# Autodesk Inventor assembly: MS-1
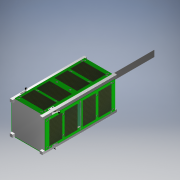
[picture p0: Inventor's stored thumbnail of the model, 180x180]
Saved by Autodesk Inventor 2022.3 (Build 263350000, 350)
## iProperties
Created: 2021-04-30
Part Number: MS-1
Document SubType Name: Assembly
Designer: Bowen O'Steen
Mass: 1447.72 g
Surface Area: 6988.67 cm^2
Volume: 630.884 cm^3
Density: 2.29475 g/cm^3
Author: Bowen O'Steen
## Documents named in this file (13)
- C:\Users\gwhen\OneDrive\Documents\Vault\Engineering Data\MemeSat\Assembly\MS-1.iam
- C:\Users\gwhen\OneDrive\Documents\Vault\Engineering Data\MemeSat\Assembly\boardstack.iam
- C:\Users\gwhen\OneDrive\Documents\Vault\Engineering Data\MemeSat\Assembly\FR-01assembled.iam
- C:\Users\gwhen\OneDrive\Documents\Vault\Engineering Data\MemeSat\Assembly\FR-04assembled.iam
- C:\Users\gwhen\OneDrive\Documents\Vault\Engineering Data\MemeSat\Assembly\FR-02assembled.iam
- C:\Users\gwhen\OneDrive\Documents\Vault\Engineering Data\MemeSat\Assembly\FR-03assembled.iam
- C:\Users\gwhen\OneDrive\Documents\Vault\Engineering Data\MemeSat\Assembly\FR-05assembled.iam
- C:\Users\gwhen\OneDrive\Documents\Vault\Engineering Data\MemeSat\Assembly\FR-06assembled.iam
- C:\Users\gwhen\OneDrive\Desktop\Vault\Designs\MEMESat\MemeSat\Engineering Data\MemeSat\Fasteners\92949A106_18-8 Stainless Steel Button Head Hex Drive Screw.ipt
- C:\Users\gwhen\OneDrive\Desktop\Vault\Designs\MEMESat\MemeSat\Engineering Data\MemeSat\Switches\ss-01gl2.ipt
- C:\Users\gwhen\OneDrive\Desktop\Vault\Designs\MEMESat\MemeSat\Engineering Data\MemeSat\Fasteners\92095A455_Button Head Hex Drive Screw.ipt
- C:\Users\gwhen\OneDrive\Desktop\Vault\Designs\MEMESat\MemeSat\Engineering Data\MemeSat\Fasteners\91828A111_18-8 Stainless Steel Hex Nut.ipt
- C:\Users\gwhen\OneDrive\Desktop\Vault\Designs\MEMESat\MemeSat\Engineering Data\MemeSat\Fasteners\90730A005.ipt
## Components (135 placed, 12 different names)
1. FR-01assembled:1 [sub-assembly] — Mate:1, Mate:2, Flush:1, Mate:3, Mate:4, Mate:5, Mate:6, Mate:7, Mate:8, Mate:13, Mate:14, Mate:15, Mate:16, Mate:47, Mate:49
2. FR-02assembled:1 [sub-assembly] — Mate:9, Mate:10, Mate:11, Mate:12, Mate:17, Mate:25, Mate:35, Mate:37, Mate:43, Mate:64, Mate:65, Mate:66, Mate:67, Mate:68, Mate:69, Mate:70, Mate:71, Mate:72, Mate:73, Mate:74, Mate:75, Mate:76, Mate:77, Mate:78, Mate:79, Mate:362, Mate:363, Mate:364, Mate:365, Mate:370, Mate:371, Mate:372, Mate:373, Mate:374, Mate:377, Mate:378, Mate:379, Mate:380, Mate:381, Mate:382, Mate:383
3. FR-03assembled:1 [sub-assembly] — Mate:6, Mate:7, Mate:8, Mate:19, Mate:20, Mate:21, Mate:22, Mate:23, Mate:24, Mate:26, Mate:59, Mate:60, Mate:61, Mate:160, Mate:161, Mate:162, Mate:163, Mate:164, Mate:165, Mate:166, Mate:167, Mate:229, Mate:230, Mate:231, Mate:244, Mate:245, Mate:270, Mate:271, Mate:302, Mate:303, Mate:308, Mate:309, Mate:320, Mate:322, Mate:334, Mate:335, Mate:358, Mate:359
4. FR-04assembled:1 [sub-assembly] — Mate:3, Mate:4, Mate:5, Mate:9, Mate:10, Mate:11, Mate:27, Mate:28, Mate:29, Mate:30, Mate:31, Mate:32, Mate:33, Mate:34, Mate:152, Mate:153, Mate:154, Mate:155, Mate:156, Mate:157, Mate:158, Mate:159, Mate:209, Mate:211, Mate:232, Mate:233, Mate:234, Mate:261, Mate:262, Mate:276, Mate:277, Mate:304, Mate:305, Mate:306, Mate:307, Mate:318, Mate:319, Mate:343, Mate:345, Mate:354, Mate:355
5. FR-05assembled:1 [sub-assembly] — Mate:15, Mate:16, Mate:17, Mate:36, Mate:38, Mate:39, Mate:40, Mate:41, Mate:42, Mate:51, Mate:52, Mate:53, Mate:54, Mate:57, Mate:144, Mate:145, Mate:146, Mate:147, Mate:148, Mate:149, Mate:150, Mate:151, Mate:225, Mate:235, Mate:236, Mate:237, Mate:241, Mate:274, Mate:275, Mate:298, Mate:299, Mate:300, Mate:301, Mate:314, Mate:315, Mate:330, Mate:331, Mate:346, Mate:347
6. FR-06assembled:1 [sub-assembly] — Mate:12, Mate:13, Mate:14, Mate:44, Mate:45, Mate:46, Mate:48, Mate:50, Mate:168, Mate:169, Mate:170, Mate:171, Mate:172, Mate:173, Mate:174, Mate:175, Mate:213, Mate:215, Mate:226, Mate:227, Mate:228, Mate:242, Mate:243, Mate:272, Mate:273, Mate:310, Mate:311, Mate:312, Mate:313, Mate:316, Mate:317, Mate:332, Mate:333, Mate:348, Mate:349
7. boardstack:1 [sub-assembly] — Mate:55, Mate:56, Mate:57, Mate:58, Mate:62, Mate:63, Mate:96, Mate:97, Mate:98, Mate:99, Mate:100, Mate:101, Mate:102, Mate:103, Mate:104, Mate:105, Mate:106, Mate:107, Mate:108, Mate:109, Mate:110, Mate:111, Mate:208, Mate:210, Mate:212, Mate:214, Mate:278, Mate:279, Mate:280, Mate:281, Mate:282, Mate:283, Mate:284, Mate:285
8. 92949A106_18-8 Stainless Steel Button Head Hex Drive Screw:2 — Mate:21, Mate:22
9. 92949A106_18-8 Stainless Steel Button Head Hex Drive Screw:3 — Mate:19, Mate:20
10. 92949A106_18-8 Stainless Steel Button Head Hex Drive Screw:4 — Mate:23, Mate:24
11. 92949A106_18-8 Stainless Steel Button Head Hex Drive Screw:5 — Mate:47, Mate:48
12. 92949A106_18-8 Stainless Steel Button Head Hex Drive Screw:6 — Mate:25, Mate:26
13. 92949A106_18-8 Stainless Steel Button Head Hex Drive Screw:7 — Mate:27, Mate:28
14. 92949A106_18-8 Stainless Steel Button Head Hex Drive Screw:8 — Mate:31, Mate:32
15. 92949A106_18-8 Stainless Steel Button Head Hex Drive Screw:9 — Mate:33, Mate:34
16. 92949A106_18-8 Stainless Steel Button Head Hex Drive Screw:10 — Mate:29, Mate:30
17. 92949A106_18-8 Stainless Steel Button Head Hex Drive Screw:11 — Mate:35, Mate:36
18. 92949A106_18-8 Stainless Steel Button Head Hex Drive Screw:12 — Mate:39, Mate:40
19. 92949A106_18-8 Stainless Steel Button Head Hex Drive Screw:13 — Mate:37, Mate:38
20. 92949A106_18-8 Stainless Steel Button Head Hex Drive Screw:14 — Mate:41, Mate:42
21. 92949A106_18-8 Stainless Steel Button Head Hex Drive Screw:15 — Mate:43, Mate:44
22. 92949A106_18-8 Stainless Steel Button Head Hex Drive Screw:16 — Mate:45, Mate:46
23. 92949A106_18-8 Stainless Steel Button Head Hex Drive Screw:17 — Mate:49, Mate:50
24. 92949A106_18-8 Stainless Steel Button Head Hex Drive Screw:18 — Mate:58, Mate:61, Mate:62
25. 92949A106_18-8 Stainless Steel Button Head Hex Drive Screw:19 — Mate:59, Mate:60, Mate:63
26. 92949A106_18-8 Stainless Steel Button Head Hex Drive Screw:20 — Mate:51, Mate:52, Mate:55
27. 92949A106_18-8 Stainless Steel Button Head Hex Drive Screw:21 — Mate:53, Mate:54, Mate:56
28. 92949A106_18-8 Stainless Steel Button Head Hex Drive Screw:22 — Mate:67, Mate:71
29. 92949A106_18-8 Stainless Steel Button Head Hex Drive Screw:23 — Mate:64, Mate:68
30. 92949A106_18-8 Stainless Steel Button Head Hex Drive Screw:24 — Mate:65, Mate:69, Mate:375
31. 92949A106_18-8 Stainless Steel Button Head Hex Drive Screw:25 — Mate:66, Mate:70, Mate:376
32. 92949A106_18-8 Stainless Steel Button Head Hex Drive Screw:26 — Mate:75, Mate:76, Mate:368
33. 92949A106_18-8 Stainless Steel Button Head Hex Drive Screw:27 — Mate:74, Mate:79, Mate:367
34. 92949A106_18-8 Stainless Steel Button Head Hex Drive Screw:28 — Mate:72, Mate:78, Mate:366
35. 92949A106_18-8 Stainless Steel Button Head Hex Drive Screw:29 — Mate:73, Mate:77, Mate:369
36. 92949A106_18-8 Stainless Steel Button Head Hex Drive Screw:30 — Mate:96, Mate:97
37. 92949A106_18-8 Stainless Steel Button Head Hex Drive Screw:31 — Mate:98, Mate:99
38. 92949A106_18-8 Stainless Steel Button Head Hex Drive Screw:32 — Mate:100, Mate:101
39. 92949A106_18-8 Stainless Steel Button Head Hex Drive Screw:33 — Mate:102, Mate:103
40. 92949A106_18-8 Stainless Steel Button Head Hex Drive Screw:34 — Mate:108, Mate:109
41. 92949A106_18-8 Stainless Steel Button Head Hex Drive Screw:35 — Mate:110, Mate:111
42. 92949A106_18-8 Stainless Steel Button Head Hex Drive Screw:36 — Mate:104, Mate:105
43. 92949A106_18-8 Stainless Steel Button Head Hex Drive Screw:37 — Mate:106, Mate:107
44. 92949A106_18-8 Stainless Steel Button Head Hex Drive Screw:38 — Mate:147, Mate:150, Mate:353
45. 92949A106_18-8 Stainless Steel Button Head Hex Drive Screw:39 — Mate:146, Mate:151, Mate:352
46. 92949A106_18-8 Stainless Steel Button Head Hex Drive Screw:40 — Mate:145, Mate:149, Mate:337
47. 92949A106_18-8 Stainless Steel Button Head Hex Drive Screw:41 — Mate:144, Mate:148, Mate:339
48. 92949A106_18-8 Stainless Steel Button Head Hex Drive Screw:42 — Mate:155, Mate:156, Mate:357
49. 92949A106_18-8 Stainless Steel Button Head Hex Drive Screw:43 — Mate:154, Mate:157, Mate:356
50. 92949A106_18-8 Stainless Steel Button Head Hex Drive Screw:44 — Mate:153, Mate:158, Mate:344
51. 92949A106_18-8 Stainless Steel Button Head Hex Drive Screw:45 — Mate:152, Mate:159, Mate:338
52. 92949A106_18-8 Stainless Steel Button Head Hex Drive Screw:46 — Mate:160, Mate:165, Mate:342
53. 92949A106_18-8 Stainless Steel Button Head Hex Drive Screw:47 — Mate:161, Mate:166, Mate:341
54. 92949A106_18-8 Stainless Steel Button Head Hex Drive Screw:48 — Mate:162, Mate:167, Mate:361
55. 92949A106_18-8 Stainless Steel Button Head Hex Drive Screw:49 — Mate:163, Mate:164, Mate:360
56. 92949A106_18-8 Stainless Steel Button Head Hex Drive Screw:50 — Mate:170, Mate:173, Mate:350
57. 92949A106_18-8 Stainless Steel Button Head Hex Drive Screw:51 — Mate:171, Mate:172, Mate:351
58. 92949A106_18-8 Stainless Steel Button Head Hex Drive Screw:52 — Mate:168, Mate:175, Mate:336
59. 92949A106_18-8 Stainless Steel Button Head Hex Drive Screw:53 — Mate:169, Mate:174, Mate:340
60. 92949A106_18-8 Stainless Steel Button Head Hex Drive Screw:54 — Mate:210, Mate:211
61. 92949A106_18-8 Stainless Steel Button Head Hex Drive Screw:55 — Mate:208, Mate:209
62. 92949A106_18-8 Stainless Steel Button Head Hex Drive Screw:56 — Mate:214, Mate:215
63. 92949A106_18-8 Stainless Steel Button Head Hex Drive Screw:57 — Mate:212, Mate:213
64. ss-01gl2:1 — Mate:232, Mate:233, Mate:234, Mate:263, Mate:264, Mate:265, Mate:266
65. ss-01gl2:2 — Mate:226, Mate:227, Mate:228, Mate:247, Mate:248, Mate:253, Mate:255
66. ss-01gl2:3 — Mate:225, Mate:235, Mate:236, Mate:238, Mate:239, Mate:246, Mate:252
67. ss-01gl2:4 — Mate:229, Mate:230, Mate:231, Mate:249, Mate:250, Mate:257, Mate:259
68. 91828A111_18-8 Stainless Steel Hex Nut:1 — Mate:239, Mate:240
69. 92095A455_Button Head Hex Drive Screw:1 — Mate:237, Mate:238, Mate:240
70. 91828A111_18-8 Stainless Steel Hex Nut:2 — Mate:253, Mate:254
71. 92095A455_Button Head Hex Drive Screw:2 — Mate:241, Mate:246, Mate:251
72. 91828A111_18-8 Stainless Steel Hex Nut:3 — Mate:255, Mate:256
73. 92095A455_Button Head Hex Drive Screw:3 — Mate:244, Mate:249, Mate:258
74. 91828A111_18-8 Stainless Steel Hex Nut:4 — Mate:251, Mate:252
75. 92095A455_Button Head Hex Drive Screw:4 — Mate:242, Mate:247, Mate:256
76. 91828A111_18-8 Stainless Steel Hex Nut:5 — Mate:257, Mate:258
77. 92095A455_Button Head Hex Drive Screw:5 — Mate:243, Mate:248, Mate:254
78. 91828A111_18-8 Stainless Steel Hex Nut:6 — Mate:259, Mate:260
79. 92095A455_Button Head Hex Drive Screw:6 — Mate:262, Mate:266, Mate:267
80. 91828A111_18-8 Stainless Steel Hex Nut:7 — Mate:263, Mate:267
81. 92095A455_Button Head Hex Drive Screw:7 — Mate:245, Mate:250, Mate:260
82. 91828A111_18-8 Stainless Steel Hex Nut:8 — Mate:264, Mate:268
83. 92095A455_Button Head Hex Drive Screw:8 — Mate:261, Mate:265, Mate:268
84. 92949A106_18-8 Stainless Steel Button Head Hex Drive Screw:58 — Mate:277, Mate:278
85. 92949A106_18-8 Stainless Steel Button Head Hex Drive Screw:59 — Mate:275, Mate:280
86. 92949A106_18-8 Stainless Steel Button Head Hex Drive Screw:60 — Mate:272, Mate:283
87. 92949A106_18-8 Stainless Steel Button Head Hex Drive Screw:61 — Mate:270, Mate:284
88. 92949A106_18-8 Stainless Steel Button Head Hex Drive Screw:62 — Mate:276, Mate:279
89. 92949A106_18-8 Stainless Steel Button Head Hex Drive Screw:63 — Mate:271, Mate:285
90. 92949A106_18-8 Stainless Steel Button Head Hex Drive Screw:64 — Mate:274, Mate:281
91. 92949A106_18-8 Stainless Steel Button Head Hex Drive Screw:65 — Mate:273, Mate:282
92. 92949A106_18-8 Stainless Steel Button Head Hex Drive Screw:71 — Mate:300, Mate:301, Mate:326
93. 92949A106_18-8 Stainless Steel Button Head Hex Drive Screw:72 — Mate:298, Mate:299, Mate:327
94. 92949A106_18-8 Stainless Steel Button Head Hex Drive Screw:74 — Mate:302, Mate:309, Mate:321
95. 92949A106_18-8 Stainless Steel Button Head Hex Drive Screw:75 — Mate:303, Mate:308, Mate:323
96. 92949A106_18-8 Stainless Steel Button Head Hex Drive Screw:76 — Mate:304, Mate:307, Mate:325
97. 92949A106_18-8 Stainless Steel Button Head Hex Drive Screw:77 — Mate:305, Mate:306, Mate:324
98. 92949A106_18-8 Stainless Steel Button Head Hex Drive Screw:78 — Mate:312, Mate:313, Mate:329
99. 92949A106_18-8 Stainless Steel Button Head Hex Drive Screw:79 — Mate:310, Mate:311, Mate:328
100. 90730A005:1 — Mate:316, Mate:328
101. 90730A005:2 — Mate:318, Mate:325
102. 90730A005:3 — Mate:317, Mate:329
103. 90730A005:4 — Mate:320, Mate:321
104. 90730A005:5 — Mate:319, Mate:324
105. 90730A005:6 — Mate:322, Mate:323
106. 90730A005:7 — Mate:314, Mate:326
107. 90730A005:8 — Mate:315, Mate:327
108. 90730A005:9 — Mate:343, Mate:344
109. 90730A005:10 — Mate:333, Mate:340
110. 90730A005:11 — Mate:334, Mate:341
111. 90730A005:12 — Mate:338, Mate:345
112. 90730A005:13 — Mate:330, Mate:337
113. 90730A005:14 — Mate:331, Mate:339
114. 90730A005:15 — Mate:335, Mate:342
115. 90730A005:16 — Mate:332, Mate:336
116. 90730A005:17 — Mate:349, Mate:351
117. 90730A005:18 — Mate:347, Mate:352
118. 90730A005:19 — Mate:346, Mate:353
119. 90730A005:20 — Mate:348, Mate:350
120. 90730A005:21 — Mate:359, Mate:360
121. 90730A005:22 — Mate:354, Mate:357
122. 90730A005:23 — Mate:358, Mate:361
123. 90730A005:24 — Mate:355, Mate:356
124. 90730A005:25 — Mate:362, Mate:366
125. 90730A005:26 — Mate:363, Mate:367
126. 90730A005:27 — Mate:364, Mate:369
127. 90730A005:28 — Mate:365, Mate:368
128. 90730A005:29 — Mate:370, Mate:376
129. 90730A005:30 — Mate:372, Mate:375
130. 90730A005:31 — Mate:371, Mate:377
131. 90730A005:32 — Mate:373, Mate:374
132. 92949A106_18-8 Stainless Steel Button Head Hex Drive Screw:80 — Mate:378, Mate:380, Mate:384
133. 92949A106_18-8 Stainless Steel Button Head Hex Drive Screw:81 — Mate:379, Mate:381, Mate:385
134. 90730A005:33 — Mate:382, Mate:384
135. 90730A005:34 — Mate:383, Mate:385
## Relationships (283: Mate 282, Flush 1)
- Mate:1: FR-01assembled:1
- Mate:2: FR-01assembled:1
- Flush:1: FR-01assembled:1
- Mate:3: FR-01assembled:1 ↔ FR-04assembled:1
- Mate:4: FR-01assembled:1 ↔ FR-04assembled:1
- Mate:5: FR-01assembled:1 ↔ FR-04assembled:1
- Mate:6: FR-01assembled:1 ↔ FR-03assembled:1
- Mate:7: FR-01assembled:1 ↔ FR-03assembled:1
- Mate:8: FR-01assembled:1 ↔ FR-03assembled:1
- Mate:9: FR-02assembled:1 ↔ FR-04assembled:1
- Mate:10: FR-02assembled:1 ↔ FR-04assembled:1
- Mate:11: FR-02assembled:1 ↔ FR-04assembled:1
- Mate:12: FR-02assembled:1 ↔ FR-06assembled:1
- Mate:13: FR-01assembled:1 ↔ FR-06assembled:1
- Mate:14: FR-01assembled:1 ↔ FR-06assembled:1
- Mate:15: FR-01assembled:1 ↔ FR-05assembled:1
- Mate:16: FR-01assembled:1 ↔ FR-05assembled:1
- Mate:17: FR-02assembled:1 ↔ FR-05assembled:1
- Mate:19: FR-03assembled:1 ↔ 92949A106_18-8 Stainless Steel Button Head Hex Drive Screw:3
- Mate:20: FR-03assembled:1 ↔ 92949A106_18-8 Stainless Steel Button Head Hex Drive Screw:3
- Mate:21: FR-03assembled:1 ↔ 92949A106_18-8 Stainless Steel Button Head Hex Drive Screw:2
- Mate:22: FR-03assembled:1 ↔ 92949A106_18-8 Stainless Steel Button Head Hex Drive Screw:2
- Mate:23: FR-03assembled:1 ↔ 92949A106_18-8 Stainless Steel Button Head Hex Drive Screw:4
- Mate:24: FR-03assembled:1 ↔ 92949A106_18-8 Stainless Steel Button Head Hex Drive Screw:4
- Mate:25: FR-02assembled:1 ↔ 92949A106_18-8 Stainless Steel Button Head Hex Drive Screw:6
- Mate:26: FR-03assembled:1 ↔ 92949A106_18-8 Stainless Steel Button Head Hex Drive Screw:6
- Mate:27: FR-04assembled:1 ↔ 92949A106_18-8 Stainless Steel Button Head Hex Drive Screw:7
- Mate:28: FR-04assembled:1 ↔ 92949A106_18-8 Stainless Steel Button Head Hex Drive Screw:7
- Mate:29: FR-04assembled:1 ↔ 92949A106_18-8 Stainless Steel Button Head Hex Drive Screw:10
- Mate:30: FR-04assembled:1 ↔ 92949A106_18-8 Stainless Steel Button Head Hex Drive Screw:10
- Mate:31: FR-04assembled:1 ↔ 92949A106_18-8 Stainless Steel Button Head Hex Drive Screw:8
- Mate:32: FR-04assembled:1 ↔ 92949A106_18-8 Stainless Steel Button Head Hex Drive Screw:8
- Mate:33: FR-04assembled:1 ↔ 92949A106_18-8 Stainless Steel Button Head Hex Drive Screw:9
- Mate:34: FR-04assembled:1 ↔ 92949A106_18-8 Stainless Steel Button Head Hex Drive Screw:9
- Mate:35: FR-02assembled:1 ↔ 92949A106_18-8 Stainless Steel Button Head Hex Drive Screw:11
- Mate:36: FR-05assembled:1 ↔ 92949A106_18-8 Stainless Steel Button Head Hex Drive Screw:11
- Mate:37: FR-02assembled:1 ↔ 92949A106_18-8 Stainless Steel Button Head Hex Drive Screw:13
- Mate:38: FR-05assembled:1 ↔ 92949A106_18-8 Stainless Steel Button Head Hex Drive Screw:13
- Mate:39: FR-05assembled:1 ↔ 92949A106_18-8 Stainless Steel Button Head Hex Drive Screw:12
- Mate:40: FR-05assembled:1 ↔ 92949A106_18-8 Stainless Steel Button Head Hex Drive Screw:12
- Mate:41: FR-05assembled:1 ↔ 92949A106_18-8 Stainless Steel Button Head Hex Drive Screw:14
- Mate:42: FR-05assembled:1 ↔ 92949A106_18-8 Stainless Steel Button Head Hex Drive Screw:14
- Mate:43: FR-02assembled:1 ↔ 92949A106_18-8 Stainless Steel Button Head Hex Drive Screw:15
- Mate:44: FR-06assembled:1 ↔ 92949A106_18-8 Stainless Steel Button Head Hex Drive Screw:15
- Mate:45: FR-06assembled:1 ↔ 92949A106_18-8 Stainless Steel Button Head Hex Drive Screw:16
- Mate:46: FR-06assembled:1 ↔ 92949A106_18-8 Stainless Steel Button Head Hex Drive Screw:16
- Mate:47: FR-01assembled:1 ↔ 92949A106_18-8 Stainless Steel Button Head Hex Drive Screw:5
- Mate:48: FR-06assembled:1 ↔ 92949A106_18-8 Stainless Steel Button Head Hex Drive Screw:5
- Mate:49: FR-01assembled:1 ↔ 92949A106_18-8 Stainless Steel Button Head Hex Drive Screw:17
- Mate:50: FR-06assembled:1 ↔ 92949A106_18-8 Stainless Steel Button Head Hex Drive Screw:17
- Mate:51: FR-05assembled:1 ↔ 92949A106_18-8 Stainless Steel Button Head Hex Drive Screw:20
- Mate:52: FR-05assembled:1 ↔ 92949A106_18-8 Stainless Steel Button Head Hex Drive Screw:20
- Mate:53: FR-05assembled:1 ↔ 92949A106_18-8 Stainless Steel Button Head Hex Drive Screw:21
- Mate:54: FR-05assembled:1 ↔ 92949A106_18-8 Stainless Steel Button Head Hex Drive Screw:21
- Mate:55: boardstack:1 ↔ 92949A106_18-8 Stainless Steel Button Head Hex Drive Screw:20
- Mate:56: boardstack:1 ↔ 92949A106_18-8 Stainless Steel Button Head Hex Drive Screw:21
- Mate:57: FR-05assembled:1 ↔ boardstack:1
- Mate:58: boardstack:1 ↔ 92949A106_18-8 Stainless Steel Button Head Hex Drive Screw:18
- Mate:59: FR-03assembled:1 ↔ 92949A106_18-8 Stainless Steel Button Head Hex Drive Screw:19
- Mate:60: FR-03assembled:1 ↔ 92949A106_18-8 Stainless Steel Button Head Hex Drive Screw:19
- Mate:61: FR-03assembled:1 ↔ 92949A106_18-8 Stainless Steel Button Head Hex Drive Screw:18
- Mate:62: boardstack:1 ↔ 92949A106_18-8 Stainless Steel Button Head Hex Drive Screw:18
- Mate:63: boardstack:1 ↔ 92949A106_18-8 Stainless Steel Button Head Hex Drive Screw:19
- Mate:64: FR-02assembled:1 ↔ 92949A106_18-8 Stainless Steel Button Head Hex Drive Screw:23
- Mate:65: FR-02assembled:1 ↔ 92949A106_18-8 Stainless Steel Button Head Hex Drive Screw:24
- Mate:66: FR-02assembled:1 ↔ 92949A106_18-8 Stainless Steel Button Head Hex Drive Screw:25
- Mate:67: FR-02assembled:1 ↔ 92949A106_18-8 Stainless Steel Button Head Hex Drive Screw:22
- Mate:68: FR-02assembled:1 ↔ 92949A106_18-8 Stainless Steel Button Head Hex Drive Screw:23
- Mate:69: FR-02assembled:1 ↔ 92949A106_18-8 Stainless Steel Button Head Hex Drive Screw:24
- Mate:70: FR-02assembled:1 ↔ 92949A106_18-8 Stainless Steel Button Head Hex Drive Screw:25
- Mate:71: FR-02assembled:1 ↔ 92949A106_18-8 Stainless Steel Button Head Hex Drive Screw:22
- Mate:72: FR-02assembled:1 ↔ 92949A106_18-8 Stainless Steel Button Head Hex Drive Screw:28
- Mate:73: FR-02assembled:1 ↔ 92949A106_18-8 Stainless Steel Button Head Hex Drive Screw:29
- Mate:74: FR-02assembled:1 ↔ 92949A106_18-8 Stainless Steel Button Head Hex Drive Screw:27
- Mate:75: FR-02assembled:1 ↔ 92949A106_18-8 Stainless Steel Button Head Hex Drive Screw:26
- Mate:76: FR-02assembled:1 ↔ 92949A106_18-8 Stainless Steel Button Head Hex Drive Screw:26
- Mate:77: FR-02assembled:1 ↔ 92949A106_18-8 Stainless Steel Button Head Hex Drive Screw:29
- Mate:78: FR-02assembled:1 ↔ 92949A106_18-8 Stainless Steel Button Head Hex Drive Screw:28
- Mate:79: FR-02assembled:1 ↔ 92949A106_18-8 Stainless Steel Button Head Hex Drive Screw:27
- Mate:96: boardstack:1 ↔ 92949A106_18-8 Stainless Steel Button Head Hex Drive Screw:30
- Mate:97: boardstack:1 ↔ 92949A106_18-8 Stainless Steel Button Head Hex Drive Screw:30
- Mate:98: boardstack:1 ↔ 92949A106_18-8 Stainless Steel Button Head Hex Drive Screw:31
- Mate:99: boardstack:1 ↔ 92949A106_18-8 Stainless Steel Button Head Hex Drive Screw:31
- Mate:100: boardstack:1 ↔ 92949A106_18-8 Stainless Steel Button Head Hex Drive Screw:32
- Mate:101: boardstack:1 ↔ 92949A106_18-8 Stainless Steel Button Head Hex Drive Screw:32
- Mate:102: boardstack:1 ↔ 92949A106_18-8 Stainless Steel Button Head Hex Drive Screw:33
- Mate:103: boardstack:1 ↔ 92949A106_18-8 Stainless Steel Button Head Hex Drive Screw:33
- Mate:104: boardstack:1 ↔ 92949A106_18-8 Stainless Steel Button Head Hex Drive Screw:36
- Mate:105: boardstack:1 ↔ 92949A106_18-8 Stainless Steel Button Head Hex Drive Screw:36
- Mate:106: boardstack:1 ↔ 92949A106_18-8 Stainless Steel Button Head Hex Drive Screw:37
- Mate:107: boardstack:1 ↔ 92949A106_18-8 Stainless Steel Button Head Hex Drive Screw:37
- Mate:108: boardstack:1 ↔ 92949A106_18-8 Stainless Steel Button Head Hex Drive Screw:34
- Mate:109: boardstack:1 ↔ 92949A106_18-8 Stainless Steel Button Head Hex Drive Screw:34
- Mate:110: boardstack:1 ↔ 92949A106_18-8 Stainless Steel Button Head Hex Drive Screw:35
- Mate:111: boardstack:1 ↔ 92949A106_18-8 Stainless Steel Button Head Hex Drive Screw:35
- Mate:144: FR-05assembled:1 ↔ 92949A106_18-8 Stainless Steel Button Head Hex Drive Screw:41
- Mate:145: FR-05assembled:1 ↔ 92949A106_18-8 Stainless Steel Button Head Hex Drive Screw:40
- Mate:146: FR-05assembled:1 ↔ 92949A106_18-8 Stainless Steel Button Head Hex Drive Screw:39
- Mate:147: FR-05assembled:1 ↔ 92949A106_18-8 Stainless Steel Button Head Hex Drive Screw:38
- Mate:148: FR-05assembled:1 ↔ 92949A106_18-8 Stainless Steel Button Head Hex Drive Screw:41
- Mate:149: FR-05assembled:1 ↔ 92949A106_18-8 Stainless Steel Button Head Hex Drive Screw:40
- Mate:150: FR-05assembled:1 ↔ 92949A106_18-8 Stainless Steel Button Head Hex Drive Screw:38
- Mate:151: FR-05assembled:1 ↔ 92949A106_18-8 Stainless Steel Button Head Hex Drive Screw:39
- Mate:152: FR-04assembled:1 ↔ 92949A106_18-8 Stainless Steel Button Head Hex Drive Screw:45
- Mate:153: FR-04assembled:1 ↔ 92949A106_18-8 Stainless Steel Button Head Hex Drive Screw:44
- Mate:154: FR-04assembled:1 ↔ 92949A106_18-8 Stainless Steel Button Head Hex Drive Screw:43
- Mate:155: FR-04assembled:1 ↔ 92949A106_18-8 Stainless Steel Button Head Hex Drive Screw:42
- Mate:156: FR-04assembled:1 ↔ 92949A106_18-8 Stainless Steel Button Head Hex Drive Screw:42
- Mate:157: FR-04assembled:1 ↔ 92949A106_18-8 Stainless Steel Button Head Hex Drive Screw:43
- Mate:158: FR-04assembled:1 ↔ 92949A106_18-8 Stainless Steel Button Head Hex Drive Screw:44
- Mate:159: FR-04assembled:1 ↔ 92949A106_18-8 Stainless Steel Button Head Hex Drive Screw:45
- Mate:160: FR-03assembled:1 ↔ 92949A106_18-8 Stainless Steel Button Head Hex Drive Screw:46
- Mate:161: FR-03assembled:1 ↔ 92949A106_18-8 Stainless Steel Button Head Hex Drive Screw:47
- Mate:162: FR-03assembled:1 ↔ 92949A106_18-8 Stainless Steel Button Head Hex Drive Screw:48
- Mate:163: FR-03assembled:1 ↔ 92949A106_18-8 Stainless Steel Button Head Hex Drive Screw:49
- Mate:164: FR-03assembled:1 ↔ 92949A106_18-8 Stainless Steel Button Head Hex Drive Screw:49
- Mate:165: FR-03assembled:1 ↔ 92949A106_18-8 Stainless Steel Button Head Hex Drive Screw:46
- Mate:166: FR-03assembled:1 ↔ 92949A106_18-8 Stainless Steel Button Head Hex Drive Screw:47
- Mate:167: FR-03assembled:1 ↔ 92949A106_18-8 Stainless Steel Button Head Hex Drive Screw:48
- Mate:168: FR-06assembled:1 ↔ 92949A106_18-8 Stainless Steel Button Head Hex Drive Screw:52
- Mate:169: FR-06assembled:1 ↔ 92949A106_18-8 Stainless Steel Button Head Hex Drive Screw:53
- Mate:170: FR-06assembled:1 ↔ 92949A106_18-8 Stainless Steel Button Head Hex Drive Screw:50
- Mate:171: FR-06assembled:1 ↔ 92949A106_18-8 Stainless Steel Button Head Hex Drive Screw:51
- Mate:172: FR-06assembled:1 ↔ 92949A106_18-8 Stainless Steel Button Head Hex Drive Screw:51
- Mate:173: FR-06assembled:1 ↔ 92949A106_18-8 Stainless Steel Button Head Hex Drive Screw:50
- Mate:174: FR-06assembled:1 ↔ 92949A106_18-8 Stainless Steel Button Head Hex Drive Screw:53
- Mate:175: FR-06assembled:1 ↔ 92949A106_18-8 Stainless Steel Button Head Hex Drive Screw:52
- Mate:208: boardstack:1 ↔ 92949A106_18-8 Stainless Steel Button Head Hex Drive Screw:55
- Mate:209: FR-04assembled:1 ↔ 92949A106_18-8 Stainless Steel Button Head Hex Drive Screw:55
- Mate:210: boardstack:1 ↔ 92949A106_18-8 Stainless Steel Button Head Hex Drive Screw:54
- Mate:211: FR-04assembled:1 ↔ 92949A106_18-8 Stainless Steel Button Head Hex Drive Screw:54
- Mate:212: boardstack:1 ↔ 92949A106_18-8 Stainless Steel Button Head Hex Drive Screw:57
- Mate:213: FR-06assembled:1 ↔ 92949A106_18-8 Stainless Steel Button Head Hex Drive Screw:57
- Mate:214: boardstack:1 ↔ 92949A106_18-8 Stainless Steel Button Head Hex Drive Screw:56
- Mate:215: FR-06assembled:1 ↔ 92949A106_18-8 Stainless Steel Button Head Hex Drive Screw:56
- Mate:225: FR-05assembled:1 ↔ ss-01gl2:3
- Mate:226: FR-06assembled:1 ↔ ss-01gl2:2
- Mate:227: FR-06assembled:1 ↔ ss-01gl2:2
- Mate:228: FR-06assembled:1 ↔ ss-01gl2:2
- Mate:229: FR-03assembled:1 ↔ ss-01gl2:4
- Mate:230: FR-03assembled:1 ↔ ss-01gl2:4
- Mate:231: FR-03assembled:1 ↔ ss-01gl2:4
- Mate:232: FR-04assembled:1 ↔ ss-01gl2:1
- Mate:233: FR-04assembled:1 ↔ ss-01gl2:1
- Mate:234: FR-04assembled:1 ↔ ss-01gl2:1
- Mate:235: FR-05assembled:1 ↔ ss-01gl2:3
- Mate:236: FR-05assembled:1 ↔ ss-01gl2:3
- Mate:237: FR-05assembled:1 ↔ 92095A455_Button Head Hex Drive Screw:1
- Mate:238: ss-01gl2:3 ↔ 92095A455_Button Head Hex Drive Screw:1
- Mate:239: ss-01gl2:3 ↔ 91828A111_18-8 Stainless Steel Hex Nut:1
- Mate:240: 91828A111_18-8 Stainless Steel Hex Nut:1 ↔ 92095A455_Button Head Hex Drive Screw:1
- Mate:241: FR-05assembled:1 ↔ 92095A455_Button Head Hex Drive Screw:2
- Mate:242: FR-06assembled:1 ↔ 92095A455_Button Head Hex Drive Screw:4
- Mate:243: FR-06assembled:1 ↔ 92095A455_Button Head Hex Drive Screw:5
- Mate:244: FR-03assembled:1 ↔ 92095A455_Button Head Hex Drive Screw:3
- Mate:245: FR-03assembled:1 ↔ 92095A455_Button Head Hex Drive Screw:7
- Mate:246: ss-01gl2:3 ↔ 92095A455_Button Head Hex Drive Screw:2
- Mate:247: ss-01gl2:2 ↔ 92095A455_Button Head Hex Drive Screw:4
- Mate:248: ss-01gl2:2 ↔ 92095A455_Button Head Hex Drive Screw:5
- Mate:249: ss-01gl2:4 ↔ 92095A455_Button Head Hex Drive Screw:3
- Mate:250: ss-01gl2:4 ↔ 92095A455_Button Head Hex Drive Screw:7
- Mate:251: 92095A455_Button Head Hex Drive Screw:2 ↔ 91828A111_18-8 Stainless Steel Hex Nut:4
- Mate:252: ss-01gl2:3 ↔ 91828A111_18-8 Stainless Steel Hex Nut:4
- Mate:253: ss-01gl2:2 ↔ 91828A111_18-8 Stainless Steel Hex Nut:2
- Mate:254: 91828A111_18-8 Stainless Steel Hex Nut:2 ↔ 92095A455_Button Head Hex Drive Screw:5
- Mate:255: ss-01gl2:2 ↔ 91828A111_18-8 Stainless Steel Hex Nut:3
- Mate:256: 91828A111_18-8 Stainless Steel Hex Nut:3 ↔ 92095A455_Button Head Hex Drive Screw:4
- Mate:257: ss-01gl2:4 ↔ 91828A111_18-8 Stainless Steel Hex Nut:5
- Mate:258: 92095A455_Button Head Hex Drive Screw:3 ↔ 91828A111_18-8 Stainless Steel Hex Nut:5
- Mate:259: ss-01gl2:4 ↔ 91828A111_18-8 Stainless Steel Hex Nut:6
- Mate:260: 91828A111_18-8 Stainless Steel Hex Nut:6 ↔ 92095A455_Button Head Hex Drive Screw:7
- Mate:261: FR-04assembled:1 ↔ 92095A455_Button Head Hex Drive Screw:8
- Mate:262: FR-04assembled:1 ↔ 92095A455_Button Head Hex Drive Screw:6
- Mate:263: ss-01gl2:1 ↔ 91828A111_18-8 Stainless Steel Hex Nut:7
- Mate:264: ss-01gl2:1 ↔ 91828A111_18-8 Stainless Steel Hex Nut:8
- Mate:265: ss-01gl2:1 ↔ 92095A455_Button Head Hex Drive Screw:8
- Mate:266: ss-01gl2:1 ↔ 92095A455_Button Head Hex Drive Screw:6
- Mate:267: 92095A455_Button Head Hex Drive Screw:6 ↔ 91828A111_18-8 Stainless Steel Hex Nut:7
- Mate:268: 91828A111_18-8 Stainless Steel Hex Nut:8 ↔ 92095A455_Button Head Hex Drive Screw:8
- Mate:270: FR-03assembled:1 ↔ 92949A106_18-8 Stainless Steel Button Head Hex Drive Screw:61
- Mate:271: FR-03assembled:1 ↔ 92949A106_18-8 Stainless Steel Button Head Hex Drive Screw:63
- Mate:272: FR-06assembled:1 ↔ 92949A106_18-8 Stainless Steel Button Head Hex Drive Screw:60
- Mate:273: FR-06assembled:1 ↔ 92949A106_18-8 Stainless Steel Button Head Hex Drive Screw:65
- Mate:274: FR-05assembled:1 ↔ 92949A106_18-8 Stainless Steel Button Head Hex Drive Screw:64
- Mate:275: FR-05assembled:1 ↔ 92949A106_18-8 Stainless Steel Button Head Hex Drive Screw:59
- Mate:276: FR-04assembled:1 ↔ 92949A106_18-8 Stainless Steel Button Head Hex Drive Screw:62
- Mate:277: FR-04assembled:1 ↔ 92949A106_18-8 Stainless Steel Button Head Hex Drive Screw:58
- Mate:278: boardstack:1 ↔ 92949A106_18-8 Stainless Steel Button Head Hex Drive Screw:58
- Mate:279: boardstack:1 ↔ 92949A106_18-8 Stainless Steel Button Head Hex Drive Screw:62
- Mate:280: boardstack:1 ↔ 92949A106_18-8 Stainless Steel Button Head Hex Drive Screw:59
- Mate:281: boardstack:1 ↔ 92949A106_18-8 Stainless Steel Button Head Hex Drive Screw:64
- Mate:282: boardstack:1 ↔ 92949A106_18-8 Stainless Steel Button Head Hex Drive Screw:65
- Mate:283: boardstack:1 ↔ 92949A106_18-8 Stainless Steel Button Head Hex Drive Screw:60
- Mate:284: boardstack:1 ↔ 92949A106_18-8 Stainless Steel Button Head Hex Drive Screw:61
- Mate:285: boardstack:1 ↔ 92949A106_18-8 Stainless Steel Button Head Hex Drive Screw:63
- Mate:298: FR-05assembled:1 ↔ 92949A106_18-8 Stainless Steel Button Head Hex Drive Screw:72
- Mate:299: FR-05assembled:1 ↔ 92949A106_18-8 Stainless Steel Button Head Hex Drive Screw:72
- Mate:300: FR-05assembled:1 ↔ 92949A106_18-8 Stainless Steel Button Head Hex Drive Screw:71
- Mate:301: FR-05assembled:1 ↔ 92949A106_18-8 Stainless Steel Button Head Hex Drive Screw:71
- Mate:302: FR-03assembled:1 ↔ 92949A106_18-8 Stainless Steel Button Head Hex Drive Screw:74
- Mate:303: FR-03assembled:1 ↔ 92949A106_18-8 Stainless Steel Button Head Hex Drive Screw:75
- Mate:304: FR-04assembled:1 ↔ 92949A106_18-8 Stainless Steel Button Head Hex Drive Screw:76
- Mate:305: FR-04assembled:1 ↔ 92949A106_18-8 Stainless Steel Button Head Hex Drive Screw:77
- Mate:306: FR-04assembled:1 ↔ 92949A106_18-8 Stainless Steel Button Head Hex Drive Screw:77
- Mate:307: FR-04assembled:1 ↔ 92949A106_18-8 Stainless Steel Button Head Hex Drive Screw:76
- Mate:308: FR-03assembled:1 ↔ 92949A106_18-8 Stainless Steel Button Head Hex Drive Screw:75
- Mate:309: FR-03assembled:1 ↔ 92949A106_18-8 Stainless Steel Button Head Hex Drive Screw:74
- Mate:310: FR-06assembled:1 ↔ 92949A106_18-8 Stainless Steel Button Head Hex Drive Screw:79
- Mate:311: FR-06assembled:1 ↔ 92949A106_18-8 Stainless Steel Button Head Hex Drive Screw:79
- Mate:312: FR-06assembled:1 ↔ 92949A106_18-8 Stainless Steel Button Head Hex Drive Screw:78
- Mate:313: FR-06assembled:1 ↔ 92949A106_18-8 Stainless Steel Button Head Hex Drive Screw:78
- Mate:314: FR-05assembled:1 ↔ 90730A005:7
- Mate:315: FR-05assembled:1 ↔ 90730A005:8
- Mate:316: FR-06assembled:1 ↔ 90730A005:1
- Mate:317: FR-06assembled:1 ↔ 90730A005:3
- Mate:318: FR-04assembled:1 ↔ 90730A005:2
- Mate:319: FR-04assembled:1 ↔ 90730A005:5
- Mate:320: FR-03assembled:1 ↔ 90730A005:4
- Mate:321: 92949A106_18-8 Stainless Steel Button Head Hex Drive Screw:74 ↔ 90730A005:4
- Mate:322: FR-03assembled:1 ↔ 90730A005:6
- Mate:323: 92949A106_18-8 Stainless Steel Button Head Hex Drive Screw:75 ↔ 90730A005:6
- Mate:324: 92949A106_18-8 Stainless Steel Button Head Hex Drive Screw:77 ↔ 90730A005:5
- Mate:325: 92949A106_18-8 Stainless Steel Button Head Hex Drive Screw:76 ↔ 90730A005:2
- Mate:326: 92949A106_18-8 Stainless Steel Button Head Hex Drive Screw:71 ↔ 90730A005:7
- Mate:327: 92949A106_18-8 Stainless Steel Button Head Hex Drive Screw:72 ↔ 90730A005:8
- Mate:328: 92949A106_18-8 Stainless Steel Button Head Hex Drive Screw:79 ↔ 90730A005:1
- Mate:329: 92949A106_18-8 Stainless Steel Button Head Hex Drive Screw:78 ↔ 90730A005:3
- Mate:330: FR-05assembled:1 ↔ 90730A005:13
- Mate:331: FR-05assembled:1 ↔ 90730A005:14
- Mate:332: FR-06assembled:1 ↔ 90730A005:16
- Mate:333: FR-06assembled:1 ↔ 90730A005:10
- Mate:334: FR-03assembled:1 ↔ 90730A005:11
- Mate:335: FR-03assembled:1 ↔ 90730A005:15
- Mate:336: 92949A106_18-8 Stainless Steel Button Head Hex Drive Screw:52 ↔ 90730A005:16
- Mate:337: 92949A106_18-8 Stainless Steel Button Head Hex Drive Screw:40 ↔ 90730A005:13
- Mate:338: 92949A106_18-8 Stainless Steel Button Head Hex Drive Screw:45 ↔ 90730A005:12
- Mate:339: 92949A106_18-8 Stainless Steel Button Head Hex Drive Screw:41 ↔ 90730A005:14
- Mate:340: 92949A106_18-8 Stainless Steel Button Head Hex Drive Screw:53 ↔ 90730A005:10
- Mate:341: 92949A106_18-8 Stainless Steel Button Head Hex Drive Screw:47 ↔ 90730A005:11
- Mate:342: 92949A106_18-8 Stainless Steel Button Head Hex Drive Screw:46 ↔ 90730A005:15
- Mate:343: FR-04assembled:1 ↔ 90730A005:9
- Mate:344: 92949A106_18-8 Stainless Steel Button Head Hex Drive Screw:44 ↔ 90730A005:9
- Mate:345: FR-04assembled:1 ↔ 90730A005:12
- Mate:346: FR-05assembled:1 ↔ 90730A005:19
- Mate:347: FR-05assembled:1 ↔ 90730A005:18
- Mate:348: FR-06assembled:1 ↔ 90730A005:20
- Mate:349: FR-06assembled:1 ↔ 90730A005:17
- Mate:350: 92949A106_18-8 Stainless Steel Button Head Hex Drive Screw:50 ↔ 90730A005:20
- Mate:351: 92949A106_18-8 Stainless Steel Button Head Hex Drive Screw:51 ↔ 90730A005:17
- Mate:352: 92949A106_18-8 Stainless Steel Button Head Hex Drive Screw:39 ↔ 90730A005:18
- Mate:353: 92949A106_18-8 Stainless Steel Button Head Hex Drive Screw:38 ↔ 90730A005:19
- Mate:354: FR-04assembled:1 ↔ 90730A005:22
- Mate:355: FR-04assembled:1 ↔ 90730A005:24
- Mate:356: 92949A106_18-8 Stainless Steel Button Head Hex Drive Screw:43 ↔ 90730A005:24
- Mate:357: 92949A106_18-8 Stainless Steel Button Head Hex Drive Screw:42 ↔ 90730A005:22
- Mate:358: FR-03assembled:1 ↔ 90730A005:23
- Mate:359: FR-03assembled:1 ↔ 90730A005:21
- Mate:360: 92949A106_18-8 Stainless Steel Button Head Hex Drive Screw:49 ↔ 90730A005:21
- Mate:361: 92949A106_18-8 Stainless Steel Button Head Hex Drive Screw:48 ↔ 90730A005:23
- Mate:362: FR-02assembled:1 ↔ 90730A005:25
- Mate:363: FR-02assembled:1 ↔ 90730A005:26
- Mate:364: FR-02assembled:1 ↔ 90730A005:27
- Mate:365: FR-02assembled:1 ↔ 90730A005:28
- Mate:366: 92949A106_18-8 Stainless Steel Button Head Hex Drive Screw:28 ↔ 90730A005:25
- Mate:367: 92949A106_18-8 Stainless Steel Button Head Hex Drive Screw:27 ↔ 90730A005:26
- Mate:368: 92949A106_18-8 Stainless Steel Button Head Hex Drive Screw:26 ↔ 90730A005:28
- Mate:369: 92949A106_18-8 Stainless Steel Button Head Hex Drive Screw:29 ↔ 90730A005:27
- Mate:370: FR-02assembled:1 ↔ 90730A005:29
- Mate:371: FR-02assembled:1 ↔ 90730A005:31
- Mate:372: FR-02assembled:1 ↔ 90730A005:30
- Mate:373: FR-02assembled:1 ↔ 90730A005:32
- Mate:374: FR-02assembled:1 ↔ 90730A005:32
- Mate:375: 92949A106_18-8 Stainless Steel Button Head Hex Drive Screw:24 ↔ 90730A005:30
- Mate:376: 92949A106_18-8 Stainless Steel Button Head Hex Drive Screw:25 ↔ 90730A005:29
- Mate:377: FR-02assembled:1 ↔ 90730A005:31
- Mate:378: FR-02assembled:1 ↔ 92949A106_18-8 Stainless Steel Button Head Hex Drive Screw:80
- Mate:379: FR-02assembled:1 ↔ 92949A106_18-8 Stainless Steel Button Head Hex Drive Screw:81
- Mate:380: FR-02assembled:1 ↔ 92949A106_18-8 Stainless Steel Button Head Hex Drive Screw:80
- Mate:381: FR-02assembled:1 ↔ 92949A106_18-8 Stainless Steel Button Head Hex Drive Screw:81
- Mate:382: FR-02assembled:1 ↔ 90730A005:33
- Mate:383: FR-02assembled:1 ↔ 90730A005:34
- Mate:384: 92949A106_18-8 Stainless Steel Button Head Hex Drive Screw:80 ↔ 90730A005:33
- Mate:385: 92949A106_18-8 Stainless Steel Button Head Hex Drive Screw:81 ↔ 90730A005:34
